# Autodesk Inventor assembly: Worm-Drive-Gearbox-16to1
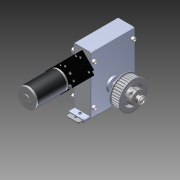
[picture p0: Inventor's stored thumbnail of the model, 180x180]
Saved by Autodesk Inventor 2014 (Build 180170000, 170)
## iProperties
Created: 2014-01-18
Part Number: Worm-Drive-Gearbox-16to1
Document SubType Name: Assembly
Designer: Michael
Author: Mark
Title: Worm Drive Gearbox 16to1.STEP
Description: STEP AP214
Creation Date: 2012-01-19
Sending System: SolidWorks 2010
Preprocessor: SwSTEP 2.0
Author: Michael
## Documents named in this file (27)
- C:\Users\Michael\Documents\GitHub\2014buildCAD\new collector mount\Worm-Drive-Gearbox-16to1.iam
- C:\Users\Michael\Documents\GitHub\2014buildCAD\Imported Components\Worm-Drive-Gearbox-16to1\FR6ZZ Bearing.ipt
- C:\Users\Michael\Documents\GitHub\2014buildCAD\Imported Components\Worm-Drive-Gearbox-16to1\Socket Head Cap Screw_AI_HX-SHCS 0.19-32x0.375x0.375-C.ipt
- C:\Users\Michael\Documents\GitHub\2014buildCAD\Imported Components\Worm-Drive-Gearbox-16to1\washer 0.25_Preferred Narrow FW 0.25.ipt
- C:\Users\Michael\Documents\GitHub\2014buildCAD\Imported Components\Worm-Drive-Gearbox-16to1\Motor mount.ipt
- C:\Users\Michael\Documents\GitHub\2014buildCAD\Imported Components\Worm-Drive-Gearbox-16to1\BHCS 0.25-20x0.625_SBHCSCREW 0.25-20x0.625-HX-C.ipt
- C:\Users\Michael\Documents\GitHub\2014buildCAD\Imported Components\Worm-Drive-Gearbox-16to1\500 hex to 8mm adapter.ipt
- C:\Users\Michael\Documents\GitHub\2014buildCAD\Imported Components\Worm-Drive-Gearbox-16to1\10-32 Nylock Nut 1_90631A411.ipt
- C:\Users\Michael\Documents\GitHub\2014buildCAD\Imported Components\Worm-Drive-Gearbox-16to1\LH Helical gear 12DP 32T 10HA 14.5PA 0.5FW_Inch - LH Helical gear 12DP 32T 10HA 14.5PA 0.5FW ---32N3.0H2.0L0.5N.ipt
- C:\Users\Michael\Documents\GitHub\2014buildCAD\Imported Components\Worm-Drive-Gearbox-16to1\SHCS 10-32x1.75_HX-SHCS 0.19-32x1.75x0.875-C.ipt
- C:\Users\Michael\Documents\GitHub\2014buildCAD\Imported Components\Worm-Drive-Gearbox-16to1\worm shaft.ipt
- C:\Users\Michael\Documents\GitHub\2014buildCAD\Imported Components\Worm-Drive-Gearbox-16to1\worm.ipt
- C:\Users\Michael\Documents\GitHub\2014buildCAD\Imported Components\Worm-Drive-Gearbox-16to1\worm spacer.ipt
- C:\Users\Michael\Documents\GitHub\2014buildCAD\Imported Components\Worm-Drive-Gearbox-16to1\End plate.ipt
- C:\Users\Michael\Documents\GitHub\2014buildCAD\Imported Components\Worm-Drive-Gearbox-16to1\o Plate.ipt
- C:\Users\Michael\Documents\GitHub\2014buildCAD\Imported Components\Worm-Drive-Gearbox-16to1\8mm spacer.ipt
- C:\Users\Michael\Documents\GitHub\2014buildCAD\Imported Components\Worm-Drive-Gearbox-16to1\worm gear ring.ipt
- C:\Users\Michael\Documents\GitHub\2014buildCAD\Imported Components\Worm-Drive-Gearbox-16to1\FR8ZZ Bearing.ipt
- C:\Users\Michael\Documents\GitHub\2014buildCAD\Imported Components\Worm-Drive-Gearbox-16to1\encoder bracket.ipt
- C:\Users\Michael\Documents\GitHub\2014buildCAD\Imported Components\Worm-Drive-Gearbox-16to1\PIN  0.1875x.75_SPS 0.1875x0.75.ipt
- C:\Users\Michael\Documents\GitHub\2014buildCAD\Imported Components\Worm-Drive-Gearbox-16to1\output shaft.ipt
- C:\Users\Michael\Documents\GitHub\2014buildCAD\Imported Components\Worm-Drive-Gearbox-16to1\Plate.ipt
- C:\Users\Michael\Documents\GitHub\2014buildCAD\Shooter\Shooter v1 (Defunct)\217-2 Stage Versaplanetary STEP.iam
- C:\Users\Michael\Documents\GitHub\2014buildCAD\new collector mount\Shaft Collar 1-2 in ID (6435K140).ipt
- C:\Users\Michael\Documents\GitHub\2014buildCAD\new collector mount\Spacer 2.ipt
- C:\Users\Michael\Documents\GitHub\2014buildCAD\new collector mount\mcmaster carr 32 tooth pulley (6497K81).ipt
- C:\Users\Michael\Documents\GitHub\2014buildCAD\new collector mount\Spacer for Belt.ipt
## Components (38 placed, 37 different names)
1. FR6ZZ Bearing_1
2. Socket Head Cap Screw_AI_HX-SHCS 0.19-32x0.375x0.375-C_2
3. washer 0.25_Preferred Narrow FW 0.25_3 — Mate:11
4. Socket Head Cap Screw_AI_HX-SHCS 0.19-32x0.375x0.375-C_5
5. Motor mount_6 — Mate:1, Mate:2, Mate:3
6. BHCS 0.25-20x0.625_SBHCSCREW 0.25-20x0.625-HX-C_7
7. 500 hex to 8mm adapter_8
8. 10-32 Nylock Nut 1_90631A411_9
9. LH Helical gear 12DP 32T 10HA 14.5PA 0.5FW_Inch - LH Helical gear 12DP 32T 10HA 14.5PA 0.5FW ---32N3.0H2.0L0.5N_10
10. SHCS 10-32x1.75_HX-SHCS 0.19-32x1.75x0.875-C_11
11. worm shaft_12
12. 10-32 Nylock Nut 1_90631A411_13
13. worm_14
14. SHCS 10-32x1.75_HX-SHCS 0.19-32x1.75x0.875-C_15
15. worm spacer_16
16. 10-32 Nylock Nut 1_90631A411_17
17. End plate_18
18. SHCS 10-32x1.75_HX-SHCS 0.19-32x1.75x0.875-C_19
19. worm spacer_20
20. 10-32 Nylock Nut 1_90631A411_21
21. o Plate_22
22. SHCS 10-32x1.75_HX-SHCS 0.19-32x1.75x0.875-C_23
23. 8mm spacer_24
24. worm gear ring_25
25. FR8ZZ Bearing_26
26. encoder bracket_27
27. PIN  0.1875x.75_SPS 0.1875x0.75_28
28. worm gear ring_29
29. FR8ZZ Bearing_30
30. output shaft_31 — Mate:5, Mate:9, Mate:15
31. Plate_32 — Angle:1, Mate:14, Mate:21, Mate:23
32. PIN  0.1875x.75_SPS 0.1875x0.75_33
33. 217-2 Stage Versaplanetary STEP:1 [sub-assembly] — Mate:1, Mate:2, Mate:3
34. Shaft Collar 1-2 in ID (6435K140):1 — Mate:5, Mate:11
35. Shaft Collar 1-2 in ID (6435K140):2 — Mate:9, Mate:16
36. Spacer 2:1 — Angle:1, Mate:14, Mate:22, Mate:24
37. mcmaster carr 32 tooth pulley (6497K81):1 — Mate:15, Mate:16
38. Spacer for Belt:1 — Mate:21, Mate:22, Mate:23, Mate:24
## Relationships (14: Mate 13, Angle 1)
- Mate:1: Motor mount_6 ↔ 217-2 Stage Versaplanetary STEP:1
- Mate:2: Motor mount_6 ↔ 217-2 Stage Versaplanetary STEP:1
- Mate:3: Motor mount_6 ↔ 217-2 Stage Versaplanetary STEP:1
- Mate:5: output shaft_31 ↔ Shaft Collar 1-2 in ID (6435K140):1
- Mate:9: output shaft_31 ↔ Shaft Collar 1-2 in ID (6435K140):2
- Mate:11 (6.35 mm): washer 0.25_Preferred Narrow FW 0.25_3 ↔ Shaft Collar 1-2 in ID (6435K140):1
- Angle:1 (0 deg): Plate_32 ↔ Spacer 2:1
- Mate:14: Plate_32 ↔ Spacer 2:1
- Mate:15: output shaft_31 ↔ mcmaster carr 32 tooth pulley (6497K81):1
- Mate:16: Shaft Collar 1-2 in ID (6435K140):2 ↔ mcmaster carr 32 tooth pulley (6497K81):1
- Mate:21: Plate_32 ↔ Spacer for Belt:1
- Mate:22: Spacer 2:1 ↔ Spacer for Belt:1
- Mate:23: Plate_32 ↔ Spacer for Belt:1
- Mate:24: Spacer 2:1 ↔ Spacer for Belt:1
